# Autodesk Inventor assembly: 3A.01.08.JS.Rib 8
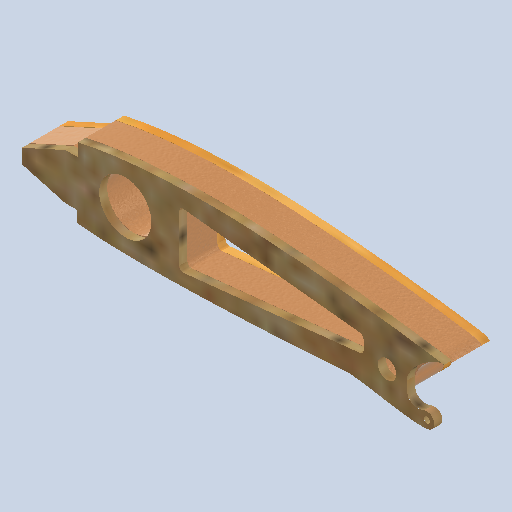
[picture p0: Inventor's stored thumbnail of the model, 512x512]
Saved by Autodesk Inventor 2025.1 (Build 291241000, 241)
## iProperties
Created: 2025-01-14
Part Number: 3A.01.08.JS.Rib 8
Document SubType Name: Assembly
Designer: johan
Author: johan
## Documents named in this file (4)
- C:\Users\johan\OneDrive - University of Bristol\CAD docs\2) Wing\2) Ribs\assemblies\3A.01.08.JS.Rib 8.iam
- C:\Users\johan\OneDrive - University of Bristol\CAD docs\2) Wing\2) Ribs\parts\Flap ribs\3P.03.08.01.JS.rib 8 ply.ipt
- C:\Users\johan\OneDrive - University of Bristol\CAD docs\2) Wing\2) Ribs\parts\Flap ribs\3P.03.08.02.JS.rib 8 foam.ipt
- C:\Users\johan\OneDrive - University of Bristol\CAD docs\2) Wing\2) Ribs\parts\Flap ribs\3P.03.08.03.JS.rib 8 hinge ply.ipt
## Components (3 placed, 3 different names)
1. 3P.03.08.01.JS.rib 8 ply:1 — Rigid:1
2. 3P.03.08.02.JS.rib 8 foam:1 — Rigid:1, Rigid:2
3. 3P.03.08.03.JS.rib 8 hinge ply:1 — Rigid:2
## Relationships (2: WeldJoint 2)
- Rigid:1 [WeldJoint]: 3P.03.08.01.JS.rib 8 ply:1 ↔ 3P.03.08.02.JS.rib 8 foam:1
- Rigid:2 [WeldJoint]: 3P.03.08.02.JS.rib 8 foam:1 ↔ 3P.03.08.03.JS.rib 8 hinge ply:1
